# Autodesk Inventor assembly: EG
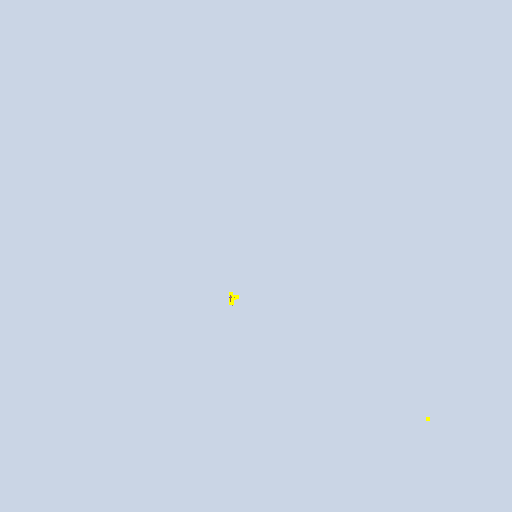
[picture p0: Inventor's stored thumbnail of the model, 512x512]
Saved by Autodesk Inventor 2024.1 (Build 281209000, 209)
## iProperties
Created: 2023-11-15
Part Number: EG
Document SubType Name: Assembly
Designer: luvag
Author: luvag
## Documents named in this file (3)
- C:\Users\luvag\Desktop\EG.iam
- C:\Users\luvag\Desktop\Assembly24.iam
- C:\Users\luvag\Desktop\pillarofdeck.ipt
## Components (5 placed, 2 different names)
1. Assembly24:1 [sub-assembly]
2. pillarofdeck:1
3. pillarofdeck:2
4. pillarofdeck:3
5. pillarofdeck:4
## Relationships (1: Mate 1)
- [Mate]: Assembly24:1 ↔ pillarofdeck:4
